# Autodesk Inventor assembly: Microdrive_Compact_withCase_Body
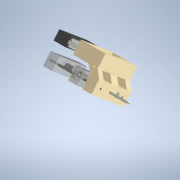
[picture p0: Inventor's stored thumbnail of the model, 180x180]
Saved by Autodesk Inventor 2020 (Build 240168000, 168)
## iProperties
Created: 2019-11-04
Part Number: Microdrive_Compact_withCase_Body
Document SubType Name: Assembly
Designer: Knowblesse
Author: Knowblesse
## Documents named in this file (4)
- C:\VCF\Microdrive\Compact\Microdrive_Compact_withCase_Body.iam
- C:\VCF\Microdrive\Compact\PCB.ipt
- C:\VCF\Microdrive\Millmax.ipt
- C:\VCF\Microdrive\Compact\Microdrive_Compact_Body.iam
## Components (3 placed, 3 different names)
1. PCB:1 — 강체:2, 강체:3
2. Millmax:1 — 강체:2
3. Microdrive_Compact_Body:1 [sub-assembly] — 강체:3
## Relationships (2: WeldJoint 2)
- 강체:2 [WeldJoint]: PCB:1 ↔ Millmax:1
- 강체:3 [WeldJoint]: PCB:1 ↔ Microdrive_Compact_Body:1
